# Autodesk Inventor assembly: MCU_PCB
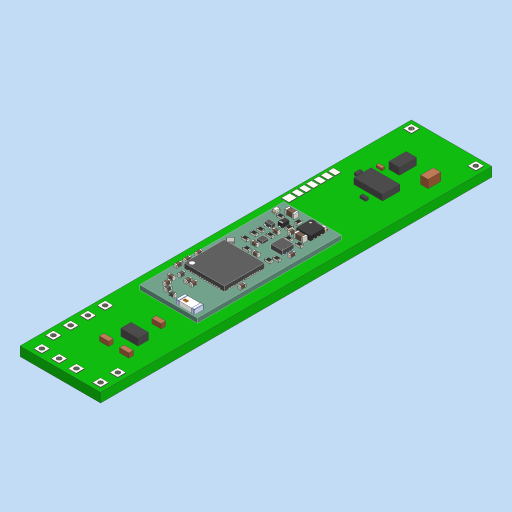
[picture p0: Inventor's stored thumbnail of the model, 512x512]
Saved by Autodesk Inventor 2024 (Build 280153000, 153)
## iProperties
Created: 2025-02-15
Part Number: MCU_PCB
Document SubType Name: Assembly
Designer: XxPan
Author: XxPan
## Documents named in this file (3)
- C:\Users\XxPan\OneDrive - McMaster University\4OI6\InkSync\case\MCU_PCB.iam
- C:\Users\XxPan\OneDrive - McMaster University\4OI6\InkSync\case\MCU_PCB.ipt
- C:\Users\XxPan\OneDrive - McMaster University\4OI6\InkSync\case\OMGS3\OMGS3.iam
## Components (2 placed, 2 different names)
1. MCU_PCB:1 — Flush:3, Mate:2, Mate:3, Mate:1, Flush:4, Flush:5
2. OMGS3:1 [sub-assembly] — Mate:1, Flush:4, Flush:5
## Relationships (6: Flush 3, Mate 3)
- Flush:3: MCU_PCB:1
- Mate:2: MCU_PCB:1
- Mate:3: MCU_PCB:1
- Mate:1: MCU_PCB:1 ↔ OMGS3:1
- Flush:4 (24.2 mm): MCU_PCB:1 ↔ OMGS3:1
- Flush:5 (2 mm): MCU_PCB:1 ↔ OMGS3:1
